# Autodesk Inventor assembly: horony_rogzito_assy
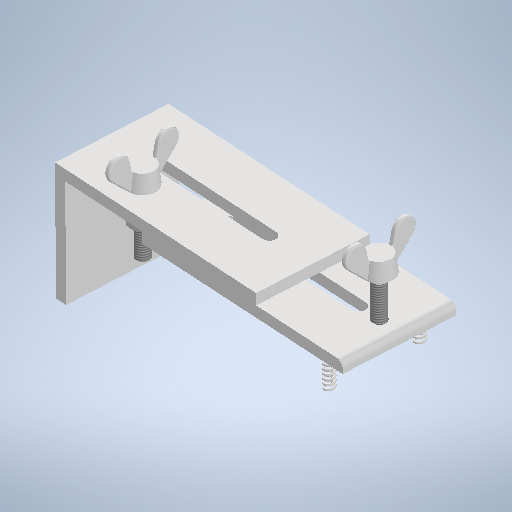
[picture p0: Inventor's stored thumbnail of the model, 512x512]
Saved by Autodesk Inventor 2025.2 (Build 292293000, 293)
## iProperties
Created: 2025-08-22
Part Number: horony_rogzito_assy
Document SubType Name: Assembly
Designer: MB
Author: MB
## Documents named in this file (5)
- C:\Users\MB\Documents\GitHub\hegesztes\horony_rogzito_assy.iam
- C:\Users\MB\Documents\GitHub\hegesztes\Horonyrogzito.ipt
- C:\Users\MB\Documents\GitHub\hegesztes\Horonyrogzito_b.ipt
- C:\Users\MB\Documents\Inventor\Content Center Files\R2025\en-US\DIN 316\DIN 316 - M6 x 30.ipt
- C:\Users\MB\Documents\Inventor\Content Center Files\R2025\en-US\ANSI B18.2.4.4M\ANSI B18.2.4.4M - M6 x 1.ipt
## Components (5 placed, 4 different names)
1. Horonyrogzito:1 — Mate:1, Flush:1, Cylindrical:2, Mate:2
2. Horonyrogzito_b:1 — Mate:1, Flush:1, Mate:3
3. DIN 316 M6 x 30:1 — Cylindrical:2
4. DIN 316 M6 x 30:2 — Cylindrical:3, Mate:3
5. Metric Hex Flange Nuts - Metric M6 x 1:1 — Cylindrical:3, Mate:2
## Relationships (6: Mate 3, CylindricalJoint 2, Flush 1)
- Mate:1: Horonyrogzito:1 ↔ Horonyrogzito_b:1
- Flush:1: Horonyrogzito:1 ↔ Horonyrogzito_b:1
- Cylindrical:2: Horonyrogzito:1 ↔ DIN 316 M6 x 30:1
- Cylindrical:3: DIN 316 M6 x 30:2 ↔ Metric Hex Flange Nuts - Metric M6 x 1:1
- Mate:2: Horonyrogzito:1 ↔ Metric Hex Flange Nuts - Metric M6 x 1:1
- Mate:3: Horonyrogzito_b:1 ↔ DIN 316 M6 x 30:2
